# Autodesk Inventor assembly: Assembly1
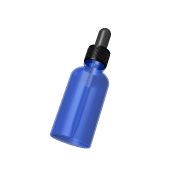
[picture p0: Inventor's stored thumbnail of the model, 180x180]
Saved by Autodesk Inventor 2015 SP2 (Build 190223200, 223)
## iProperties
Created: 2016-12-12
Part Number: Assembly1
Document SubType Name: Assembly
Designer: dsnyder
Author: dsnyder
## Documents named in this file (5)
- C:\Users\dsnyder\Documents\Personal\Temporary\EyeDropperBottle\EyeDropperBottle.iam
- C:\Users\dsnyder\Documents\Personal\Temporary\EyeDropperBottle\Bottle.ipt
- C:\Users\dsnyder\Documents\Personal\Temporary\EyeDropperBottle\Cap.ipt
- C:\Users\dsnyder\Documents\Personal\Temporary\EyeDropperBottle\Bulb.ipt
- C:\Users\dsnyder\Documents\Personal\Temporary\EyeDropperBottle\Pipette.ipt
## Components (4 placed, 4 different names)
1. Bottle:1 — Mate:2, Mate:3, Insert:2
2. Cap:1 — Mate:1, Mate:2
3. Bulb:1 — Insert:1, Mate:1, Insert:2
4. Pipette:1 — Insert:1, Mate:3
## Relationships (5: Mate 3, Insert 2)
- Insert:1 (-3.175 mm): Bulb:1 ↔ Pipette:1
- Mate:1: Cap:1 ↔ Bulb:1
- Mate:2: Bottle:1 ↔ Cap:1
- Mate:3: Bottle:1 ↔ Pipette:1
- Insert:2: Bottle:1 ↔ Bulb:1
